# Autodesk Inventor assembly: Assembly front bottom coupler + bracket
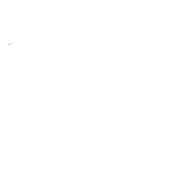
[picture p0: Inventor's stored thumbnail of the model, 180x180]
Saved by Autodesk Inventor 2020 (Build 240168000, 168)
## iProperties
Created: 2019-11-16
Part Number: Assembly front bottom coupler + bracket
Document SubType Name: Assembly
Designer: ball
Author: ball
## Documents named in this file (4)
- C:\FTC\FTC8863CAD\2019 Robot\Delivery\Assembly front bottom coupler + bracket.iam
- C:\FTC\FTC8863CAD\2019 Robot\Delivery\Front fixed bottom coupler.ipt
- C:\FTC\FTC8863CAD\2019 Robot\Delivery\Mounting Bracket Bottom.ipt
- C:\FTC\FTC8863CAD\StepLibraries\Nuts\m3 18-8 STAINLESS STL NYLON-INSERT LOCKNUT.ipt
## Components (4 placed, 3 different names)
1. Front fixed bottom coupler:1 — Flush:1, Flush:2
2. Mounting Bracket Bottom:1 — Flush:1, Flush:2, Mate:1, Mate:2
3. m3 18-8 STAINLESS STL NYLON-INSERT LOCKNUT:1 — Mate:1
4. m3 18-8 STAINLESS STL NYLON-INSERT LOCKNUT:2 — Mate:2
## Relationships (4: Flush 2, Mate 2)
- Flush:1: Front fixed bottom coupler:1 ↔ Mounting Bracket Bottom:1
- Flush:2: Front fixed bottom coupler:1 ↔ Mounting Bracket Bottom:1
- Mate:1: Mounting Bracket Bottom:1 ↔ m3 18-8 STAINLESS STL NYLON-INSERT LOCKNUT:1
- Mate:2: Mounting Bracket Bottom:1 ↔ m3 18-8 STAINLESS STL NYLON-INSERT LOCKNUT:2
